# Autodesk Inventor assembly: inner
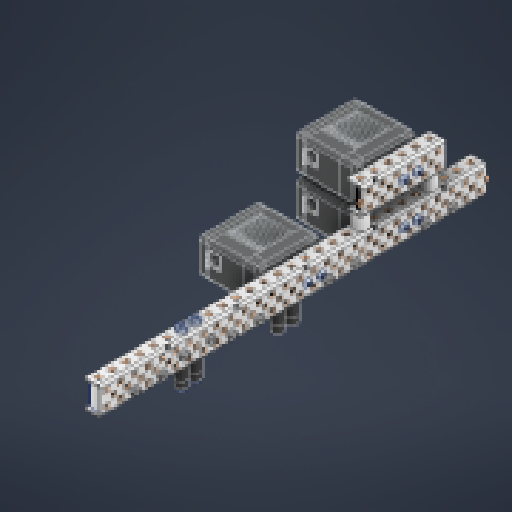
[picture p0: Inventor's stored thumbnail of the model, 512x512]
Saved by Autodesk Inventor 2024 (Build 280153000, 153)
## iProperties
Created: 2023-10-18
Part Number: inner
Document SubType Name: Assembly
Designer: Averey Ku
Author: Averey Ku
## Documents named in this file (18)
- D:\vex_robotics\hardware\cad\goated_v0.1\chassis\drivebay\inner.iam
- D:\vex_robotics\hardware\cad\VEX-CAD-Inventor-1.41\Structure\C Channel\Aluminum 1x2x1\Alu C 1x2x1x28.ipt
- D:\vex_robotics\hardware\cad\VEX-CAD-Inventor-1.41\Structure\C Channel\Aluminum 1x2x1\Alu C 1x2x1x6.ipt
- D:\vex_robotics\hardware\cad\VEX-CAD-Inventor-1.41\Structure\Standoff\Standoff .875.ipt
- D:\vex_robotics\hardware\cad\VEX-CAD-Inventor-1.41\Structure\Standoff.ipt
- D:\vex_robotics\hardware\cad\hardware\.375 OD Aluminum Spacer 0.875.ipt
- D:\vex_robotics\hardware\cad\VEX-CAD-Inventor-1.41\Electronics\Motors with Screws\SteelM-StarS.iam
- D:\vex_robotics\hardware\cad\VEX-CAD-Inventor-1.41\Electronics\Motors with Screws.iam
- D:\vex_robotics\hardware\cad\VEX-CAD-Inventor-1.41\Motion\Spacers\Spacer Nylon .500 OD\NSpacer White .500 OD x .500.ipt
- D:\vex_robotics\hardware\cad\VEX-CAD-Inventor-1.41\Motion\Spacers\Spacer Nylon .500 OD.ipt
- D:\vex_robotics\hardware\cad\VEX-CAD-Inventor-1.41\lightweight_bearing.iam
- D:\vex_robotics\hardware\cad\VEX-CAD-Inventor-1.41\Motion\Spacers\Spacer Nylon .375 OD\NSpacer .375 OD x .500.ipt
- D:\vex_robotics\hardware\cad\VEX-CAD-Inventor-1.41\Motion\Spacers\Spacer Nylon .375 OD.ipt
- D:\vex_robotics\hardware\cad\VEX-CAD-Inventor-1.41\Structure\Hardware\Nut Keps.ipt
- D:\vex_robotics\hardware\cad\VEX-CAD-Inventor-1.41\Structure\Hardware\Screw Shoulder Robosource\SScrew Shoulder Smooth 2.000 x .04.ipt
- D:\vex_robotics\hardware\cad\VEX-CAD-Inventor-1.41\Structure\Hardware\Screw Shoulder Robosource.ipt
- D:\vex_robotics\hardware\cad\VEX-CAD-Inventor-1.41\Structure\Hardware\Nut Hex.ipt
- D:\vex_robotics\hardware\cad\VEX-CAD-Inventor-1.41\Motion\Spacers\Spacer Nylon .375 OD\NSpacer .375 OD x .250.ipt
## Components (37 placed, 12 different names)
1. Alu C 1x2x1x28:1 — Insert:3, Mate:1, Insert:4, Insert:6, Mate:3, Insert:7, Insert:8, Insert:9, Mate:4, Insert:10, Mate:5, Insert:11, Mate:6, Insert:12, Mate:7, Insert:13, Insert:14, Insert:15, Insert:16, Insert:17, Insert:18, Insert:24, Insert:25, Mate:9, Insert:26, Mate:10, Insert:32, Insert:33, Insert:35, Insert:36
2. Alu C 1x2x1x6:1 — Insert:3, Mate:1, Insert:5, Mate:2
3. Standoff .875:1
4. Standoff .875:2
5. .375 OD Aluminum Spacer 0.875:1 — Insert:4
6. SteelM-StarS:1 [sub-assembly] — Insert:5, Mate:2
7. SteelM-StarS:2 [sub-assembly] — Insert:6, Mate:3
8. NSpacer White .500 OD x .500:1 — Insert:8
9. NSpacer White .500 OD x .500:2 — Insert:7
10. SteelM-StarS:3 [sub-assembly] — Insert:9, Mate:4
11. lightweight_bearing:1 [sub-assembly] — Insert:10, Mate:5, Insert:28
12. lightweight_bearing:2 [sub-assembly] — Insert:11, Mate:6, Insert:29
13. lightweight_bearing:3 [sub-assembly] — Insert:12, Mate:7, Insert:27
14. NSpacer .375 OD x .500:1 — Insert:14, Insert:21, Insert:34
15. NSpacer .375 OD x .500:2 — Insert:13, Insert:20, Insert:37
16. Nut Keps:1 — Insert:18
17. Nut Keps:2 — Insert:17
18. Nut Keps:3 — Insert:16
19. Nut Keps:4 — Insert:15
20. SScrew Shoulder Smooth 2.000 x .04:1 — Insert:20
21. SScrew Shoulder Smooth 2.000 x .04:2 — Insert:21
22. Nut Hex:1 — Insert:36
23. Nut Hex:2 — Insert:35
24. .375 OD Aluminum Spacer 0.875:2 — Insert:24
25. lightweight_bearing:4 [sub-assembly] — Insert:25, Mate:9, Insert:30
26. lightweight_bearing:5 [sub-assembly] — Insert:26, Mate:10, Insert:31
27. Nut Hex:3 — Insert:27
28. Nut Hex:4 — Insert:29
29. Nut Hex:5 — Insert:31
30. Nut Hex:6 — Insert:30
31. Nut Hex:7 — Insert:28
32. NSpacer .375 OD x .500:3 — Insert:32, Insert:39
33. NSpacer .375 OD x .500:4 — Insert:33, Insert:38
34. NSpacer .375 OD x .250:5 — Insert:34
35. NSpacer .375 OD x .250:6 — Insert:37
36. NSpacer .375 OD x .250:7 — Insert:38
37. NSpacer .375 OD x .250:8 — Insert:39
## Relationships (45: Insert 36, Mate 9)
- [Insert]: Alu C 1x2x1x6:1 ↔ Standoff .875:1
- [Insert]: Alu C 1x2x1x6:1 ↔ Standoff .875:2
- Insert:3 (12.7 mm): Alu C 1x2x1x28:1 ↔ Alu C 1x2x1x6:1
- Mate:1: Alu C 1x2x1x28:1 ↔ Alu C 1x2x1x6:1
- Insert:4: Alu C 1x2x1x28:1 ↔ .375 OD Aluminum Spacer 0.875:1
- Insert:5: Alu C 1x2x1x6:1 ↔ SteelM-StarS:1
- Mate:2: Alu C 1x2x1x6:1 ↔ SteelM-StarS:1
- Insert:6: Alu C 1x2x1x28:1 ↔ SteelM-StarS:2
- Mate:3: Alu C 1x2x1x28:1 ↔ SteelM-StarS:2
- Insert:7: Alu C 1x2x1x28:1 ↔ NSpacer White .500 OD x .500:2
- Insert:8: Alu C 1x2x1x28:1 ↔ NSpacer White .500 OD x .500:1
- Insert:9: Alu C 1x2x1x28:1 ↔ SteelM-StarS:3
- Mate:4: Alu C 1x2x1x28:1 ↔ SteelM-StarS:3
- Insert:10: Alu C 1x2x1x28:1 ↔ lightweight_bearing:1
- Mate:5: Alu C 1x2x1x28:1 ↔ lightweight_bearing:1
- Insert:11: Alu C 1x2x1x28:1 ↔ lightweight_bearing:2
- Mate:6: Alu C 1x2x1x28:1 ↔ lightweight_bearing:2
- Insert:12: Alu C 1x2x1x28:1 ↔ lightweight_bearing:3
- Mate:7: Alu C 1x2x1x28:1 ↔ lightweight_bearing:3
- Insert:13: Alu C 1x2x1x28:1 ↔ NSpacer .375 OD x .500:2
- Insert:14: Alu C 1x2x1x28:1 ↔ NSpacer .375 OD x .500:1
- Insert:15: Alu C 1x2x1x28:1 ↔ Nut Keps:4
- Insert:16: Alu C 1x2x1x28:1 ↔ Nut Keps:3
- Insert:17: Alu C 1x2x1x28:1 ↔ Nut Keps:2
- Insert:18: Alu C 1x2x1x28:1 ↔ Nut Keps:1
- Insert:20 (7.9375 mm): NSpacer .375 OD x .500:2 ↔ SScrew Shoulder Smooth 2.000 x .04:1
- Insert:21 (7.9375 mm): NSpacer .375 OD x .500:1 ↔ SScrew Shoulder Smooth 2.000 x .04:2
- Insert:24: Alu C 1x2x1x28:1 ↔ .375 OD Aluminum Spacer 0.875:2
- Insert:25: Alu C 1x2x1x28:1 ↔ lightweight_bearing:4
- Mate:9: Alu C 1x2x1x28:1 ↔ lightweight_bearing:4
- Insert:26: Alu C 1x2x1x28:1 ↔ lightweight_bearing:5
- Mate:10: Alu C 1x2x1x28:1 ↔ lightweight_bearing:5
- Insert:27 (1.27 mm): lightweight_bearing:3 ↔ Nut Hex:3
- Insert:28 (1.27 mm): lightweight_bearing:1 ↔ Nut Hex:7
- Insert:29 (1.27 mm): lightweight_bearing:2 ↔ Nut Hex:4
- Insert:30 (1.27 mm): lightweight_bearing:4 ↔ Nut Hex:6
- Insert:31 (1.27 mm): lightweight_bearing:5 ↔ Nut Hex:5
- Insert:32: Alu C 1x2x1x28:1 ↔ NSpacer .375 OD x .500:3
- Insert:33: Alu C 1x2x1x28:1 ↔ NSpacer .375 OD x .500:4
- Insert:34: NSpacer .375 OD x .500:1 ↔ NSpacer .375 OD x .250:5
- Insert:35: Alu C 1x2x1x28:1 ↔ Nut Hex:2
- Insert:36: Alu C 1x2x1x28:1 ↔ Nut Hex:1
- Insert:37: NSpacer .375 OD x .500:2 ↔ NSpacer .375 OD x .250:6
- Insert:38: NSpacer .375 OD x .500:4 ↔ NSpacer .375 OD x .250:7
- Insert:39: NSpacer .375 OD x .500:3 ↔ NSpacer .375 OD x .250:8
